# Autodesk Inventor assembly: !Hook
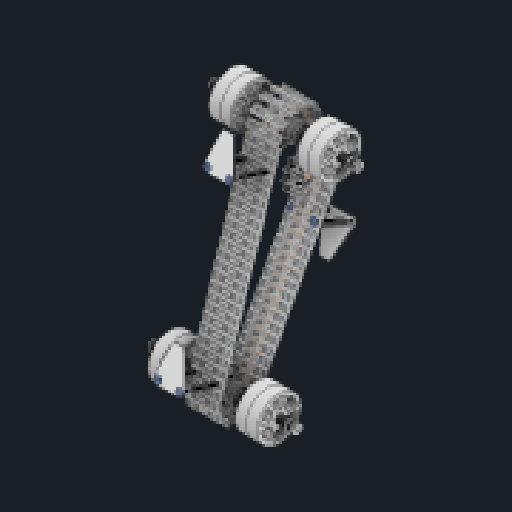
[picture p0: Inventor's stored thumbnail of the model, 512x512]
Saved by Autodesk Inventor 2025 (Build 290162000, 162)
## iProperties
Created: 2024-10-20
Part Number: !Hook
Document SubType Name: Assembly
Designer: Averey Ku
Author: Averey Ku
## Documents named in this file (11)
- D:\VEX\High Stakes\CAD\V2\Hook\!Hook.iam
- D:\VEX\High Stakes\CAD\V2\Hook\Chain.iam
- D:\VEX\High Stakes\CAD\V2\Hook\Custom Parts\Hook Gusset.ipt
- D:\VEX\High Stakes\CAD\ROBOPROS-CAD-Inventor\Structure\Standoff\Standoff .25.ipt
- D:\VEX\High Stakes\CAD\ROBOPROS-CAD-Inventor\Structure\Standoff.ipt
- D:\VEX\High Stakes\CAD\ROBOPROS-CAD-Inventor\Structure\Standoff\Standoff 1.50.ipt
- D:\VEX\High Stakes\CAD\ROBOPROS-CAD-Inventor\Structure\Hardware\Screw Shoulder Robosource\SScrew Shoulder Smooth .500 x .04.ipt
- D:\VEX\High Stakes\CAD\ROBOPROS-CAD-Inventor\Structure\Hardware\Screw Shoulder Robosource.ipt
- D:\VEX\High Stakes\CAD\ROBOPROS-CAD-Inventor\Motion\Sprockets\9P Sprocket\9P 12T Sprocket, No Insert.iam
- D:\VEX\High Stakes\CAD\ROBOPROS-CAD-Inventor\Motion\Sprockets\9P Sprocket.iam
- D:\VEX\High Stakes\CAD\V2\Hook\Roller Shaft.iam
## Components (31 placed, 7 different names)
1. Chain:1 [sub-assembly] — Insert:1, Insert:4, Insert:9, Insert:10, Insert:20, Mate:5, Insert:31, Mate:6, Mate:7, Mate:8, Mate:9
2. Roller Shaft:1 [sub-assembly] — Flush:1, Mate:7, Mate:10
3. Roller Shaft:2 [sub-assembly] — Flush:2, Mate:8
4. 9P 12T Sprocket, No Insert:1 [sub-assembly] — Mate:9, Mate:10
5. Hook Gusset:1 — Insert:3, Insert:6, Insert:7, Insert:8
6. Standoff .25:1 — Insert:5, Insert:6
7. Standoff 1.50:2 — Insert:4, Insert:5
8. Standoff .25:3 — Insert:2, Insert:3
9. Standoff 1.50:4 — Insert:1, Insert:2
10. SScrew Shoulder Smooth .500 x .04:1 — Insert:8
11. SScrew Shoulder Smooth .500 x .04:2 — Insert:7
12. SScrew Shoulder Smooth .500 x .04:3 — Insert:10
13. SScrew Shoulder Smooth .500 x .04:4 — Insert:9
14. Hook Gusset:2
15. Standoff .25:5
16. Standoff 1.50:6 — Insert:20, Insert:21
17. Standoff .25:7
18. Standoff 1.50:8 — Mate:5, Insert:22
19. SScrew Shoulder Smooth .500 x .04:5
20. SScrew Shoulder Smooth .500 x .04:6
21. SScrew Shoulder Smooth .500 x .04:8 — Insert:22
22. SScrew Shoulder Smooth .500 x .04:7 — Insert:21
23. Hook Gusset:3
24. Standoff .25:9
25. Standoff 1.50:10 — Mate:6
26. Standoff .25:11
27. Standoff 1.50:12 — Insert:31
28. SScrew Shoulder Smooth .500 x .04:9
29. SScrew Shoulder Smooth .500 x .04:10
30. SScrew Shoulder Smooth .500 x .04:11
31. SScrew Shoulder Smooth .500 x .04:12
## Relationships (36: Insert 28, Mate 6, Flush 2)
- Insert:1: Chain:1 ↔ Standoff 1.50:4
- Insert:2: Standoff .25:3 ↔ Standoff 1.50:4
- Insert:3: Hook Gusset:1 ↔ Standoff .25:3
- Insert:4: Chain:1 ↔ Standoff 1.50:2
- Insert:5: Standoff .25:1 ↔ Standoff 1.50:2
- Insert:6: Hook Gusset:1 ↔ Standoff .25:1
- Insert:7: Hook Gusset:1 ↔ SScrew Shoulder Smooth .500 x .04:2
- Insert:8: Hook Gusset:1 ↔ SScrew Shoulder Smooth .500 x .04:1
- Insert:9: Chain:1 ↔ SScrew Shoulder Smooth .500 x .04:4
- Insert:10: Chain:1 ↔ SScrew Shoulder Smooth .500 x .04:3
- [Insert]: Standoff .25:7 ↔ Standoff 1.50:8
- [Insert]: Hook Gusset:2 ↔ Standoff .25:7
- [Insert]: Standoff .25:5 ↔ Standoff 1.50:6
- [Insert]: Hook Gusset:2 ↔ Standoff .25:5
- [Insert]: Hook Gusset:2 ↔ SScrew Shoulder Smooth .500 x .04:6
- [Insert]: Hook Gusset:2 ↔ SScrew Shoulder Smooth .500 x .04:5
- Insert:20: Chain:1 ↔ Standoff 1.50:6
- Mate:5: Chain:1 ↔ Standoff 1.50:8
- Insert:21 (3.175 mm): Standoff 1.50:6 ↔ SScrew Shoulder Smooth .500 x .04:7
- Insert:22 (3.175 mm): Standoff 1.50:8 ↔ SScrew Shoulder Smooth .500 x .04:8
- [Insert]: Standoff .25:11 ↔ Standoff 1.50:12
- [Insert]: Hook Gusset:3 ↔ Standoff .25:11
- [Insert]: Standoff .25:9 ↔ Standoff 1.50:10
- [Insert]: Hook Gusset:3 ↔ Standoff .25:9
- [Insert]: Hook Gusset:3 ↔ SScrew Shoulder Smooth .500 x .04:10
- [Insert]: Hook Gusset:3 ↔ SScrew Shoulder Smooth .500 x .04:9
- [Insert] (3.175 mm): Standoff 1.50:10 ↔ SScrew Shoulder Smooth .500 x .04:11
- [Insert] (3.175 mm): Standoff 1.50:12 ↔ SScrew Shoulder Smooth .500 x .04:12
- Insert:31: Chain:1 ↔ Standoff 1.50:12
- Mate:6: Chain:1 ↔ Standoff 1.50:10
- Flush:1 (6.35 mm): Roller Shaft:1
- Mate:7: Chain:1 ↔ Roller Shaft:1
- Flush:2 (6.35 mm): Roller Shaft:2
- Mate:8: Chain:1 ↔ Roller Shaft:2
- Mate:9: Chain:1 ↔ 9P 12T Sprocket, No Insert:1
- Mate:10: Roller Shaft:1 ↔ 9P 12T Sprocket, No Insert:1
## Named parameters: d16_d1 = 0 mm, d17_d2 = 0 mm, d18_d4 = 0 mm, d19_d5 = 0 mm, d20_d6 = 0 mm, d21_d7 = 0 mm, d30_d28 = 3.175 mm, d31_d29 = 3.175 mm, d32_d16_d1 = 0 mm, d33_d17_d2 = 0 mm, d34_d18_d4 = 0 mm, d35_d19_d5 = 0 mm, d36_d20_d6 = 0 mm, d37_d21_d7 = 0 mm
